# Autodesk Inventor assembly: Mecanum_Assembly
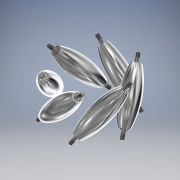
[picture p0: Inventor's stored thumbnail of the model, 180x180]
Saved by Autodesk Inventor 2018 (Build 220112000, 112)
## iProperties
Created: 2017-09-05
Part Number: Mecanum_Assembly
Document SubType Name: Assembly
Designer: P136265
Author: P136265
## Documents named in this file (4)
- C:\Users\P136265\Documents\mecanum-cad\Mecanum_Assembly.iam
- C:\Users\P136265\Documents\mecanum-cad\roller 8-19-6 bearing.ipt
- C:\Users\P136265\Documents\Inventor\Content Center Files\R2018\en-US\DIN 625 SKF(4)\DIN 625 SKF - SKF 619_8-2Z.ipt
- C:\Users\P136265\Documents\mecanum-cad\MecanumShaft.ipt
## Components (24 placed, 3 different names)
1. roller 8-19-6 bearing:1 — Mate:1, Angle:1, Mate:2
2. roller 8-19-6 bearing:2
3. roller 8-19-6 bearing:3 — Insert:1, Insert:2
4. roller 8-19-6 bearing:4 — Angle:2, Mate:3
5. roller 8-19-6 bearing:5
6. roller 8-19-6 bearing:6
7. DIN 625 SKF- with two Z shields SKF 619/8-2Z:1 — Insert:1
8. DIN 625 SKF- with two Z shields SKF 619/8-2Z:3
9. DIN 625 SKF- with two Z shields SKF 619/8-2Z:4
10. DIN 625 SKF- with two Z shields SKF 619/8-2Z:5
11. DIN 625 SKF- with two Z shields SKF 619/8-2Z:6
12. DIN 625 SKF- with two Z shields SKF 619/8-2Z:7
13. DIN 625 SKF- with two Z shields SKF 619/8-2Z:2 — Insert:2
14. DIN 625 SKF- with two Z shields SKF 619/8-2Z:8 — Flush:1
15. DIN 625 SKF- with two Z shields SKF 619/8-2Z:9
16. DIN 625 SKF- with two Z shields SKF 619/8-2Z:10
17. DIN 625 SKF- with two Z shields SKF 619/8-2Z:11
18. DIN 625 SKF- with two Z shields SKF 619/8-2Z:12
19. MecanumShaft:1 — Angle:2, Mate:3, Flush:1
20. MecanumShaft:2
21. MecanumShaft:3
22. MecanumShaft:4
23. MecanumShaft:5
24. MecanumShaft:6
## Component patterns: (6 elements, first: roller 8-19-6 bearing:1), (6 elements, first: DIN 625 SKF- with two Z shields SKF 619/8-2Z:1), (6 elements, first: DIN 625 SKF- with two Z shields SKF 619/8-2Z:2), (6 elements, first: MecanumShaft:1)
## Relationships (8: Mate 3, Angle 2, Insert 2, Flush 1)
- Mate:1 (75 mm): roller 8-19-6 bearing:1
- Angle:1 (45 deg): roller 8-19-6 bearing:1
- Mate:2: roller 8-19-6 bearing:1
- Insert:1: roller 8-19-6 bearing:3 ↔ DIN 625 SKF- with two Z shields SKF 619/8-2Z:1
- Insert:2: roller 8-19-6 bearing:3 ↔ DIN 625 SKF- with two Z shields SKF 619/8-2Z:2
- Angle:2 (0 deg): roller 8-19-6 bearing:4 ↔ MecanumShaft:1
- Mate:3: roller 8-19-6 bearing:4 ↔ MecanumShaft:1
- Flush:1 (-20 mm): DIN 625 SKF- with two Z shields SKF 619/8-2Z:8 ↔ MecanumShaft:1
